# Autodesk Inventor assembly: Upright_Assembly_V2
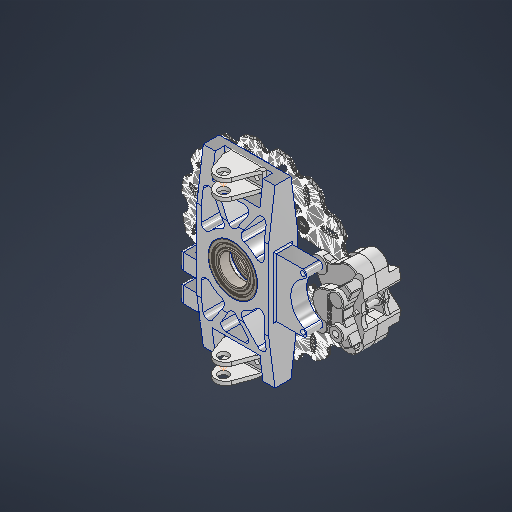
[picture p0: Inventor's stored thumbnail of the model, 512x512]
Saved by Autodesk Inventor 2026.1 (Build 301233000, 233)
## iProperties
Created: 2026-09-03
Part Number: Upright_Assembly_V2
Document SubType Name: Assembly
Designer: share
Author: share
## iProperties of the stored document MemberDocs/xP5h1hnmtLk5vqzscZ5ldh2xhLf
Created: 2026-09-03
Part Number: Upright_Assembly_V2
Document SubType Name: Assembly
Designer: share
Author: share
## iProperties of the stored document MemberDocs/xMwqub40oHcne2agnJcglx0bqGg
Created: 2026-09-03
Part Number: Upright_Assembly_V2
Document SubType Name: Assembly
Designer: share
Author: share
## Documents named in this file (13)
- C:\Users\share\OneDrive\Documents\Personal Projects\GOGO Kart\CAD\GOGO_KART_FSAE\Suspension\REAL Upright\V2\Upright_Assembly_V2.iam
- C:\Users\share\OneDrive\Documents\Personal Projects\GOGO Kart\CAD\GOGO_KART_FSAE\Suspension\REAL Upright\V2\Suspension_Upright_V2.ipt
- C:\Users\share\OneDrive\Documents\Personal Projects\GOGO Kart\CAD\GOGO_KART_FSAE\Suspension\Bearings\grainger-35hz68\grainger-35hz68\grainger-35hz68.ipt
- C:\Users\share\OneDrive\Documents\Personal Projects\GOGO Kart\CAD\GOGO_KART_FSAE\Suspension\Hardware\ALLSTAR 0.5 in Rod End Bracket (Rough).ipt
- C:\Users\share\Downloads\Brake_caliper-W-PS1_1808987814.214\Brake_caliper-W-PS1_1808987814.214\Brake_caliper-W-PS1_1808987814.214.iam
- C:\Users\share\OneDrive\Documents\Personal Projects\GOGO Kart\CAD\GOGO_KART_FSAE\Suspension\Uprights\Arashi Rear Brake Disc Rotors.ipt
- C:\Users\share\OneDrive\Documents\Personal Projects\GOGO Kart\CAD\GOGO_KART_FSAE\Suspension\hoosier-r25b-20x7-5-13-13-oz-aluminum-wheel-1.snapshot.2\Hoosier + OZ Rim.ipt
- C:\Users\share\OneDrive\Documents\Personal Projects\GOGO Kart\CAD\GOGO_KART_FSAE\Suspension\REAL Upright\V2\Spindle_CV_Flange_V2.ipt
- C:\Users\share\OneDrive\Documents\Personal Projects\GOGO Kart\CAD\GOGO_KART_FSAE\Suspension\REAL Upright\V2\Wheel_Hub_V2.ipt
- C:\Users\share\Downloads\93849A106_18-8 Stainless Steel Washer\93849A106_18-8 Stainless Steel Washer\93849A106_18-8 Stainless Steel Washer.ipt
- C:\Users\share\OneDrive\Documents\Personal Projects\GOGO Kart\CAD\GOGO_KART_FSAE\Suspension\Hardware\Lug Stud M12 X 45.ipt
- C:\Users\share\OneDrive\Documents\Personal Projects\GOGO Kart\CAD\GOGO_KART_FSAE\Suspension\Hardware\ISO 4014 - M10 x 100 - ISO.ipt
- C:\Users\share\OneDrive\Documents\Inventor\Content Center Files\R2026\en-US\ISO 4033(2)\ISO 4033 - M10 - ISO.ipt
## Components (7 placed, 5 different names)
1. Suspension_Upright_V2:1 — Flush:1, Flush:2, Flush:3, Insert:1, Insert:2, Mate:1, Insert:5, Insert:6, Insert:7, Insert:8, Insert:11, Insert:12, Insert:13, Insert:14
2. grainger-35hz68:1 — Insert:2, Mate:2
3. grainger-35hz68:2 — Insert:1
4. ALLSTAR 0.5 in Rod End Bracket (Rough):1 — Mate:1, Insert:5, Insert:6
5. ALLSTAR 0.5 in Rod End Bracket (Rough):2 — Insert:7, Insert:8
6. Brake_caliper-W-PS1_1808987814.214:1 [sub-assembly] — Mate:3, Insert:11, Insert:12, Insert:13, Insert:14
7. Arashi Rear Brake Disc Rotors:1 — Mate:2, Mate:3
## Relationships (16: Insert 10, Flush 3, Mate 3)
- Flush:1: Suspension_Upright_V2:1
- Flush:2: Suspension_Upright_V2:1
- Flush:3: Suspension_Upright_V2:1
- Insert:1: Suspension_Upright_V2:1 ↔ grainger-35hz68:2
- Insert:2: Suspension_Upright_V2:1 ↔ grainger-35hz68:1
- Mate:1: Suspension_Upright_V2:1 ↔ ALLSTAR 0.5 in Rod End Bracket (Rough):1
- Insert:5: Suspension_Upright_V2:1 ↔ ALLSTAR 0.5 in Rod End Bracket (Rough):1
- Insert:6: Suspension_Upright_V2:1 ↔ ALLSTAR 0.5 in Rod End Bracket (Rough):1
- Insert:7: Suspension_Upright_V2:1 ↔ ALLSTAR 0.5 in Rod End Bracket (Rough):2
- Insert:8: Suspension_Upright_V2:1 ↔ ALLSTAR 0.5 in Rod End Bracket (Rough):2
- Mate:2: grainger-35hz68:1 ↔ Arashi Rear Brake Disc Rotors:1
- Mate:3: Brake_caliper-W-PS1_1808987814.214:1 ↔ Arashi Rear Brake Disc Rotors:1
- Insert:11: Suspension_Upright_V2:1 ↔ Brake_caliper-W-PS1_1808987814.214:1
- Insert:12: Suspension_Upright_V2:1 ↔ Brake_caliper-W-PS1_1808987814.214:1
- Insert:13: Suspension_Upright_V2:1 ↔ Brake_caliper-W-PS1_1808987814.214:1
- Insert:14: Suspension_Upright_V2:1 ↔ Brake_caliper-W-PS1_1808987814.214:1
